# Autodesk Inventor assembly: BG201_trajan20_21
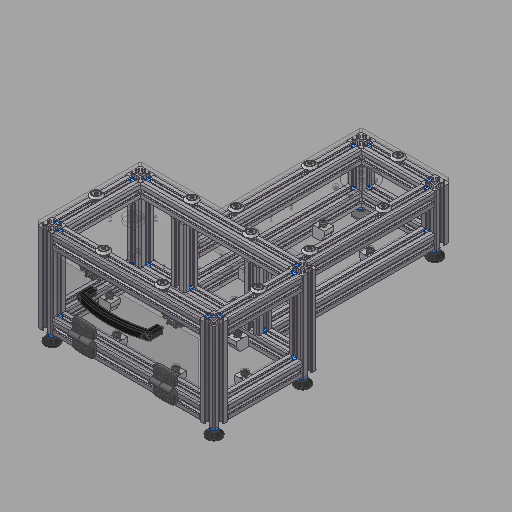
[picture p0: Inventor's stored thumbnail of the model, 512x512]
Saved by Autodesk Inventor 2022.2 (Build 262287000, 287)
## iProperties
Company: HTBLA Kaindorf
RuleStatus: InUse
Created: 2022-08-22
Part Number: BG201_trajan20_21
Project: Zeichenmaschine_v2
Material: Generisch
Description: gerüst_mit_platten
Document SubType Name: Assembly
Designer: trajan20
AfterDocNew0: iProperties-Editor_aufrufen
Author: jan
Keywords: 2021
## Documents named in this file (15)
- C:\Users\jan\Documents\DrawMachine\DrawMachineConstruction\Projekt\Zeichenmaschine_v2\BG201_trajan20_21_Zeichenmaschine_v2_gerüst_mit_platten.iam
- C:\Users\jan\Documents\DrawMachine\DrawMachineConstruction\Projekt\Zeichenmaschine_v2\BG103_trajan20_21_Zeichenmaschine_v2_Gerüst_Step_zu_Bauteil.iam
- C:\Users\jan\Documents\DrawMachine\DrawMachineConstruction\Projekt\Zeichenmaschine_v2\BT201_trajan20_21_Zeichenmaschine_v2_Hauptplatte unten.ipt
- C:\Users\jan\Documents\DrawMachine\DrawMachineConstruction\Projekt\Zeichenmaschine_v2\BT202_trajan20_21_Zeichenmaschine_v2_getriebemotor platte unten.ipt
- C:\Users\jan\Documents\DrawMachine\DrawMachineConstruction\Projekt\Zeichenmaschine_v2\BT101_trajan20_21_Zeichenmaschine_v2_Platte Stepper Motoren.ipt
- C:\Users\jan\Documents\DrawMachine\DrawMachineConstruction\Projekt\Zeichenmaschine_v2\BT102_trajan20_21_Zeichenmaschine_v2_Platte Getriebemotor.ipt
- C:\Users\jan\Documents\DrawMachine\DrawMachineConstruction\Projekt\Zeichenmaschine_v2\Normteile\de-DE\ISO 14583\ISO 14583 - M4x12-A3-70.ipt
- C:\Users\jan\Documents\DrawMachine\DrawMachineConstruction\Projekt\Zeichenmaschine_v2\step dateien\BN 603 1229915 finishing washer M5.ipt
- C:\Users\jan\Documents\DrawMachine\DrawMachineConstruction\Projekt\Zeichenmaschine_v2\Senkschraube DIN ≈965 M5x14 51305_050_014(High).ipt
- C:\Users\jan\Documents\DrawMachine\DrawMachineConstruction\Projekt\Zeichenmaschine_v2\ART 48240 - DIN 6900-1 Z0 T M4x12_0 mm - A2_Steel.ipt
- C:\Users\jan\Documents\DrawMachine\DrawMachineConstruction\Projekt\Zeichenmaschine_v2\Senkschraube DIN ≈965 M4x8 51305_040_008(High).ipt
- C:\Users\jan\Documents\DrawMachine\DrawMachineConstruction\Projekt\Zeichenmaschine_v2\BT703_trajan20_21_Zeichenmaschine_v2_Plexitür_200x80.ipt
- C:\Users\jan\Documents\DrawMachine\DrawMachineConstruction\Projekt\Zeichenmaschine_v2\Normteile\de-DE\AS 1427(03)\AS 1427 - M2 x 4(1).ipt
- C:\Users\jan\Documents\DrawMachine\DrawMachineConstruction\Projekt\Zeichenmaschine_v2\Normteile\de-DE\ISO 4762(2)\ISO 4762 - M4 x 16ISO.ipt
- C:\Users\jan\Documents\DrawMachine\DrawMachineConstruction\Projekt\Zeichenmaschine_v2\BT703_B_trajan20_21_Zeichenmaschine_v2_Griff.ipt
## Components (57 placed, 14 different names)
1. BG103_trajan20_21_Zeichenmaschine_v2_Gerüst_Step_zu_Bauteil:1 [sub-assembly] — Passend:1, Passend:2, Passend:3, Passend:4, Passend:5, Passend:6, Passend:7, Fluchtend:1, Fluchtend:2, Fluchtend:3, Passend:8, Fluchtend:4, Passend:64, Passend:65, Passend:66, Passend:67, Passend:68, Passend:69, Passend:70, Passend:71, Passend:72, Passend:73, Passend:74, Passend:75, Passend:76, Passend:77, Passend:78, Passend:79, Passend:83, Passend:85, Passend:86, Passend:87, Passend:88, Passend:89, Passend:90, Passend:91, Passend:92, Passend:93, Passend:94
2. BT201_trajan20_21_Zeichenmaschine_v2_Hauptplatte unten:1 — Passend:1, Passend:2, Passend:3, Einfügen:1, Passend:9, Passend:10, Passend:11, Passend:12, Passend:13, Passend:14, Passend:15, Passend:16, Passend:17, Passend:18
3. BT202_trajan20_21_Zeichenmaschine_v2_getriebemotor platte unten:1 — Passend:4, Passend:5, Passend:6, Passend:19, Passend:20, Passend:21, Passend:22, Passend:23, Passend:24, Passend:25, Passend:26, Passend:27, Passend:28, Passend:51, Passend:52
4. BT101_trajan20_21_Zeichenmaschine_v2_Platte Stepper Motoren:1 — Passend:7, Fluchtend:1, Fluchtend:2, Passend:29, Passend:30, Passend:31, Passend:32, Passend:33, Passend:34, Passend:35, Passend:36, Passend:37, Passend:38, Passend:39, Passend:40
5. BT102_trajan20_21_Zeichenmaschine_v2_Platte Getriebemotor:1 — Fluchtend:3, Passend:8, Fluchtend:4, Passend:41, Passend:42, Passend:43, Passend:44, Passend:45, Passend:46, Passend:47, Passend:48, Passend:49, Passend:50
6. BN 603 1229915 finishing washer M5:1 — Passend:29, Passend:30, Passend:62, Fluchtend:14
7. BN 603 1229915 finishing washer M5:2 — Passend:31, Passend:32, Passend:61, Fluchtend:13
8. BN 603 1229915 finishing washer M5:3 — Passend:33, Passend:34, Passend:60, Fluchtend:12
9. BN 603 1229915 finishing washer M5:4 — Passend:35, Passend:36, Passend:59, Fluchtend:11
10. BN 603 1229915 finishing washer M5:5 — Passend:37, Passend:38, Passend:58, Fluchtend:10
11. BN 603 1229915 finishing washer M5:6 — Passend:39, Passend:40, Passend:63, Fluchtend:15
12. BN 603 1229915 finishing washer M5:7 — Passend:41, Passend:42, Passend:54, Fluchtend:6
13. BN 603 1229915 finishing washer M5:8 — Passend:43, Passend:44, Passend:53, Fluchtend:5
14. BN 603 1229915 finishing washer M5:9 — Passend:45, Passend:46, Passend:57, Fluchtend:9
15. BN 603 1229915 finishing washer M5:10 — Passend:47, Passend:48, Passend:56, Fluchtend:8
16. BN 603 1229915 finishing washer M5:11 — Passend:49, Passend:50, Passend:55, Fluchtend:7
17. Schraube ISO 14583:2011(E) M4x12-A3-70:12 — Passend:51, Passend:52
18. Senkschraube DIN ≈965 M5x14 51305_050_014(High):1 — Passend:53, Fluchtend:5
19. Senkschraube DIN ≈965 M5x14 51305_050_014(High):2 — Passend:54, Fluchtend:6
20. Senkschraube DIN ≈965 M5x14 51305_050_014(High):3 — Passend:55, Fluchtend:7
21. Senkschraube DIN ≈965 M5x14 51305_050_014(High):4 — Passend:56, Fluchtend:8
22. Senkschraube DIN ≈965 M5x14 51305_050_014(High):5 — Passend:57, Fluchtend:9
23. Senkschraube DIN ≈965 M5x14 51305_050_014(High):6 — Passend:58, Fluchtend:10
24. Senkschraube DIN ≈965 M5x14 51305_050_014(High):7 — Passend:59, Fluchtend:11
25. Senkschraube DIN ≈965 M5x14 51305_050_014(High):8 — Passend:60, Fluchtend:12
26. Senkschraube DIN ≈965 M5x14 51305_050_014(High):9 — Passend:61, Fluchtend:13
27. Senkschraube DIN ≈965 M5x14 51305_050_014(High):10 — Passend:62, Fluchtend:14
28. Senkschraube DIN ≈965 M5x14 51305_050_014(High):11 — Passend:63, Fluchtend:15
29. ART 48240 - DIN 6900-1 Z0 T M4x12_0 mm - A2_Steel:1 — Passend:64, Passend:65
30. ART 48240 - DIN 6900-1 Z0 T M4x12_0 mm - A2_Steel:2 — Passend:66, Passend:67
31. ART 48240 - DIN 6900-1 Z0 T M4x12_0 mm - A2_Steel:3 — Passend:68, Passend:71
32. ART 48240 - DIN 6900-1 Z0 T M4x12_0 mm - A2_Steel:4 — Passend:69, Passend:70
33. Senkschraube DIN ≈965 M4x8 51305_040_008(High):1 — Passend:72, Passend:73
34. Senkschraube DIN ≈965 M4x8 51305_040_008(High):2 — Passend:74, Passend:75
35. Senkschraube DIN ≈965 M4x8 51305_040_008(High):3 — Passend:76, Passend:77
36. Senkschraube DIN ≈965 M4x8 51305_040_008(High):4 — Passend:78, Passend:79
37. BT703_trajan20_21_Zeichenmaschine_v2_Plexitür_200x80:1 — Passend:80, Passend:81, Passend:82, Passend:83, Passend:84, Passend:85, Passend:86, Passend:95, Passend:96, Passend:97
38. AS 1427 - Metrisch M2 x 4:1 — Passend:80, Passend:81
39. AS 1427 - Metrisch M2 x 4:2 — Passend:82, Passend:84
40. Senkschraube DIN ≈965 M4x8 51305_040_008(High):5 — Passend:87, Passend:93
41. Senkschraube DIN ≈965 M4x8 51305_040_008(High):6 — Passend:88, Passend:94
42. Senkschraube DIN ≈965 M4x8 51305_040_008(High):7 — Passend:89, Passend:92
43. Senkschraube DIN ≈965 M4x8 51305_040_008(High):8 — Passend:90, Passend:91
44. ISO 4762 M4 x 16:1 — Passend:98, Passend:101
45. BT703_B_trajan20_21_Zeichenmaschine_v2_Griff:1 — Passend:95, Passend:96, Passend:97, Passend:98, Passend:99, Passend:100, Passend:101
46. ISO 4762 M4 x 16:2 — Passend:99, Passend:100
47. Schraube ISO 14583:2011(E) M4x12-A3-70:1 — Einfügen:1
48. Schraube ISO 14583:2011(E) M4x12-A3-70:2 — Passend:9, Passend:10
49. Schraube ISO 14583:2011(E) M4x12-A3-70:3 — Passend:11, Passend:12
50. Schraube ISO 14583:2011(E) M4x12-A3-70:4 — Passend:13, Passend:14
51. Schraube ISO 14583:2011(E) M4x12-A3-70:5 — Passend:15, Passend:16
52. Schraube ISO 14583:2011(E) M4x12-A3-70:6 — Passend:17, Passend:18
53. Schraube ISO 14583:2011(E) M4x12-A3-70:7 — Passend:19, Passend:20
54. Schraube ISO 14583:2011(E) M4x12-A3-70:8 — Passend:21, Passend:22
55. Schraube ISO 14583:2011(E) M4x12-A3-70:9 — Passend:23, Passend:24
56. Schraube ISO 14583:2011(E) M4x12-A3-70:10 — Passend:25, Passend:26
57. Schraube ISO 14583:2011(E) M4x12-A3-70:11 — Passend:27, Passend:28
## Relationships (117: Mate 101, Flush 15, Insert 1)
- Passend:1 [Mate]: BG103_trajan20_21_Zeichenmaschine_v2_Gerüst_Step_zu_Bauteil:1 ↔ BT201_trajan20_21_Zeichenmaschine_v2_Hauptplatte unten:1
- Passend:2 [Mate]: BG103_trajan20_21_Zeichenmaschine_v2_Gerüst_Step_zu_Bauteil:1 ↔ BT201_trajan20_21_Zeichenmaschine_v2_Hauptplatte unten:1
- Passend:3 [Mate]: BG103_trajan20_21_Zeichenmaschine_v2_Gerüst_Step_zu_Bauteil:1 ↔ BT201_trajan20_21_Zeichenmaschine_v2_Hauptplatte unten:1
- Passend:4 [Mate]: BG103_trajan20_21_Zeichenmaschine_v2_Gerüst_Step_zu_Bauteil:1 ↔ BT202_trajan20_21_Zeichenmaschine_v2_getriebemotor platte unten:1
- Passend:5 [Mate]: BG103_trajan20_21_Zeichenmaschine_v2_Gerüst_Step_zu_Bauteil:1 ↔ BT202_trajan20_21_Zeichenmaschine_v2_getriebemotor platte unten:1
- Passend:6 [Mate]: BG103_trajan20_21_Zeichenmaschine_v2_Gerüst_Step_zu_Bauteil:1 ↔ BT202_trajan20_21_Zeichenmaschine_v2_getriebemotor platte unten:1
- Passend:7 [Mate]: BG103_trajan20_21_Zeichenmaschine_v2_Gerüst_Step_zu_Bauteil:1 ↔ BT101_trajan20_21_Zeichenmaschine_v2_Platte Stepper Motoren:1
- Fluchtend:1 [Flush]: BG103_trajan20_21_Zeichenmaschine_v2_Gerüst_Step_zu_Bauteil:1 ↔ BT101_trajan20_21_Zeichenmaschine_v2_Platte Stepper Motoren:1
- Fluchtend:2 [Flush]: BG103_trajan20_21_Zeichenmaschine_v2_Gerüst_Step_zu_Bauteil:1 ↔ BT101_trajan20_21_Zeichenmaschine_v2_Platte Stepper Motoren:1
- Fluchtend:3 [Flush]: BG103_trajan20_21_Zeichenmaschine_v2_Gerüst_Step_zu_Bauteil:1 ↔ BT102_trajan20_21_Zeichenmaschine_v2_Platte Getriebemotor:1
- Passend:8 [Mate]: BG103_trajan20_21_Zeichenmaschine_v2_Gerüst_Step_zu_Bauteil:1 ↔ BT102_trajan20_21_Zeichenmaschine_v2_Platte Getriebemotor:1
- Fluchtend:4 [Flush]: BG103_trajan20_21_Zeichenmaschine_v2_Gerüst_Step_zu_Bauteil:1 ↔ BT102_trajan20_21_Zeichenmaschine_v2_Platte Getriebemotor:1
- Einfügen:1 [Insert]: BT201_trajan20_21_Zeichenmaschine_v2_Hauptplatte unten:1 ↔ Schraube ISO 14583:2011(E) M4x12-A3-70:1
- Passend:9 [Mate]: BT201_trajan20_21_Zeichenmaschine_v2_Hauptplatte unten:1 ↔ Schraube ISO 14583:2011(E) M4x12-A3-70:2
- Passend:10 [Mate]: BT201_trajan20_21_Zeichenmaschine_v2_Hauptplatte unten:1 ↔ Schraube ISO 14583:2011(E) M4x12-A3-70:2
- Passend:11 [Mate]: BT201_trajan20_21_Zeichenmaschine_v2_Hauptplatte unten:1 ↔ Schraube ISO 14583:2011(E) M4x12-A3-70:3
- Passend:12 [Mate]: BT201_trajan20_21_Zeichenmaschine_v2_Hauptplatte unten:1 ↔ Schraube ISO 14583:2011(E) M4x12-A3-70:3
- Passend:13 [Mate]: BT201_trajan20_21_Zeichenmaschine_v2_Hauptplatte unten:1 ↔ Schraube ISO 14583:2011(E) M4x12-A3-70:4
- Passend:14 [Mate]: BT201_trajan20_21_Zeichenmaschine_v2_Hauptplatte unten:1 ↔ Schraube ISO 14583:2011(E) M4x12-A3-70:4
- Passend:15 [Mate]: BT201_trajan20_21_Zeichenmaschine_v2_Hauptplatte unten:1 ↔ Schraube ISO 14583:2011(E) M4x12-A3-70:5
- Passend:16 [Mate]: BT201_trajan20_21_Zeichenmaschine_v2_Hauptplatte unten:1 ↔ Schraube ISO 14583:2011(E) M4x12-A3-70:5
- Passend:17 [Mate]: BT201_trajan20_21_Zeichenmaschine_v2_Hauptplatte unten:1 ↔ Schraube ISO 14583:2011(E) M4x12-A3-70:6
- Passend:18 [Mate]: BT201_trajan20_21_Zeichenmaschine_v2_Hauptplatte unten:1 ↔ Schraube ISO 14583:2011(E) M4x12-A3-70:6
- Passend:19 [Mate]: BT202_trajan20_21_Zeichenmaschine_v2_getriebemotor platte unten:1 ↔ Schraube ISO 14583:2011(E) M4x12-A3-70:7
- Passend:20 [Mate]: BT202_trajan20_21_Zeichenmaschine_v2_getriebemotor platte unten:1 ↔ Schraube ISO 14583:2011(E) M4x12-A3-70:7
- Passend:21 [Mate]: BT202_trajan20_21_Zeichenmaschine_v2_getriebemotor platte unten:1 ↔ Schraube ISO 14583:2011(E) M4x12-A3-70:8
- Passend:22 [Mate]: BT202_trajan20_21_Zeichenmaschine_v2_getriebemotor platte unten:1 ↔ Schraube ISO 14583:2011(E) M4x12-A3-70:8
- Passend:23 [Mate]: BT202_trajan20_21_Zeichenmaschine_v2_getriebemotor platte unten:1 ↔ Schraube ISO 14583:2011(E) M4x12-A3-70:9
- Passend:24 [Mate]: BT202_trajan20_21_Zeichenmaschine_v2_getriebemotor platte unten:1 ↔ Schraube ISO 14583:2011(E) M4x12-A3-70:9
- Passend:25 [Mate]: BT202_trajan20_21_Zeichenmaschine_v2_getriebemotor platte unten:1 ↔ Schraube ISO 14583:2011(E) M4x12-A3-70:10
- Passend:26 [Mate]: BT202_trajan20_21_Zeichenmaschine_v2_getriebemotor platte unten:1 ↔ Schraube ISO 14583:2011(E) M4x12-A3-70:10
- Passend:27 [Mate]: BT202_trajan20_21_Zeichenmaschine_v2_getriebemotor platte unten:1 ↔ Schraube ISO 14583:2011(E) M4x12-A3-70:11
- Passend:28 [Mate]: BT202_trajan20_21_Zeichenmaschine_v2_getriebemotor platte unten:1 ↔ Schraube ISO 14583:2011(E) M4x12-A3-70:11
- Passend:29 [Mate]: BT101_trajan20_21_Zeichenmaschine_v2_Platte Stepper Motoren:1 ↔ BN 603 1229915 finishing washer M5:1
- Passend:30 [Mate]: BT101_trajan20_21_Zeichenmaschine_v2_Platte Stepper Motoren:1 ↔ BN 603 1229915 finishing washer M5:1
- Passend:31 [Mate]: BT101_trajan20_21_Zeichenmaschine_v2_Platte Stepper Motoren:1 ↔ BN 603 1229915 finishing washer M5:2
- Passend:32 [Mate]: BT101_trajan20_21_Zeichenmaschine_v2_Platte Stepper Motoren:1 ↔ BN 603 1229915 finishing washer M5:2
- Passend:33 [Mate]: BT101_trajan20_21_Zeichenmaschine_v2_Platte Stepper Motoren:1 ↔ BN 603 1229915 finishing washer M5:3
- Passend:34 [Mate]: BT101_trajan20_21_Zeichenmaschine_v2_Platte Stepper Motoren:1 ↔ BN 603 1229915 finishing washer M5:3
- Passend:35 [Mate]: BT101_trajan20_21_Zeichenmaschine_v2_Platte Stepper Motoren:1 ↔ BN 603 1229915 finishing washer M5:4
- Passend:36 [Mate]: BT101_trajan20_21_Zeichenmaschine_v2_Platte Stepper Motoren:1 ↔ BN 603 1229915 finishing washer M5:4
- Passend:37 [Mate]: BT101_trajan20_21_Zeichenmaschine_v2_Platte Stepper Motoren:1 ↔ BN 603 1229915 finishing washer M5:5
- Passend:38 [Mate]: BT101_trajan20_21_Zeichenmaschine_v2_Platte Stepper Motoren:1 ↔ BN 603 1229915 finishing washer M5:5
- Passend:39 [Mate]: BT101_trajan20_21_Zeichenmaschine_v2_Platte Stepper Motoren:1 ↔ BN 603 1229915 finishing washer M5:6
- Passend:40 [Mate]: BT101_trajan20_21_Zeichenmaschine_v2_Platte Stepper Motoren:1 ↔ BN 603 1229915 finishing washer M5:6
- Passend:41 [Mate]: BT102_trajan20_21_Zeichenmaschine_v2_Platte Getriebemotor:1 ↔ BN 603 1229915 finishing washer M5:7
- Passend:42 [Mate]: BT102_trajan20_21_Zeichenmaschine_v2_Platte Getriebemotor:1 ↔ BN 603 1229915 finishing washer M5:7
- Passend:43 [Mate]: BT102_trajan20_21_Zeichenmaschine_v2_Platte Getriebemotor:1 ↔ BN 603 1229915 finishing washer M5:8
- Passend:44 [Mate]: BT102_trajan20_21_Zeichenmaschine_v2_Platte Getriebemotor:1 ↔ BN 603 1229915 finishing washer M5:8
- Passend:45 [Mate]: BT102_trajan20_21_Zeichenmaschine_v2_Platte Getriebemotor:1 ↔ BN 603 1229915 finishing washer M5:9
- Passend:46 [Mate]: BT102_trajan20_21_Zeichenmaschine_v2_Platte Getriebemotor:1 ↔ BN 603 1229915 finishing washer M5:9
- Passend:47 [Mate]: BT102_trajan20_21_Zeichenmaschine_v2_Platte Getriebemotor:1 ↔ BN 603 1229915 finishing washer M5:10
- Passend:48 [Mate]: BT102_trajan20_21_Zeichenmaschine_v2_Platte Getriebemotor:1 ↔ BN 603 1229915 finishing washer M5:10
- Passend:49 [Mate]: BT102_trajan20_21_Zeichenmaschine_v2_Platte Getriebemotor:1 ↔ BN 603 1229915 finishing washer M5:11
- Passend:50 [Mate]: BT102_trajan20_21_Zeichenmaschine_v2_Platte Getriebemotor:1 ↔ BN 603 1229915 finishing washer M5:11
- Passend:51 [Mate]: BT202_trajan20_21_Zeichenmaschine_v2_getriebemotor platte unten:1 ↔ Schraube ISO 14583:2011(E) M4x12-A3-70:12
- Passend:52 [Mate]: BT202_trajan20_21_Zeichenmaschine_v2_getriebemotor platte unten:1 ↔ Schraube ISO 14583:2011(E) M4x12-A3-70:12
- Passend:53 [Mate]: BN 603 1229915 finishing washer M5:8 ↔ Senkschraube DIN ≈965 M5x14 51305_050_014(High):1
- Fluchtend:5 [Flush]: BN 603 1229915 finishing washer M5:8 ↔ Senkschraube DIN ≈965 M5x14 51305_050_014(High):1
- Passend:54 [Mate]: BN 603 1229915 finishing washer M5:7 ↔ Senkschraube DIN ≈965 M5x14 51305_050_014(High):2
- Fluchtend:6 [Flush]: BN 603 1229915 finishing washer M5:7 ↔ Senkschraube DIN ≈965 M5x14 51305_050_014(High):2
- Passend:55 [Mate]: BN 603 1229915 finishing washer M5:11 ↔ Senkschraube DIN ≈965 M5x14 51305_050_014(High):3
- Fluchtend:7 [Flush]: BN 603 1229915 finishing washer M5:11 ↔ Senkschraube DIN ≈965 M5x14 51305_050_014(High):3
- Passend:56 [Mate]: BN 603 1229915 finishing washer M5:10 ↔ Senkschraube DIN ≈965 M5x14 51305_050_014(High):4
- Fluchtend:8 [Flush]: BN 603 1229915 finishing washer M5:10 ↔ Senkschraube DIN ≈965 M5x14 51305_050_014(High):4
- Passend:57 [Mate]: BN 603 1229915 finishing washer M5:9 ↔ Senkschraube DIN ≈965 M5x14 51305_050_014(High):5
- Fluchtend:9 [Flush]: BN 603 1229915 finishing washer M5:9 ↔ Senkschraube DIN ≈965 M5x14 51305_050_014(High):5
- Passend:58 [Mate]: BN 603 1229915 finishing washer M5:5 ↔ Senkschraube DIN ≈965 M5x14 51305_050_014(High):6
- Fluchtend:10 [Flush]: BN 603 1229915 finishing washer M5:5 ↔ Senkschraube DIN ≈965 M5x14 51305_050_014(High):6
- Passend:59 [Mate]: BN 603 1229915 finishing washer M5:4 ↔ Senkschraube DIN ≈965 M5x14 51305_050_014(High):7
- Fluchtend:11 [Flush]: BN 603 1229915 finishing washer M5:4 ↔ Senkschraube DIN ≈965 M5x14 51305_050_014(High):7
- Passend:60 [Mate]: BN 603 1229915 finishing washer M5:3 ↔ Senkschraube DIN ≈965 M5x14 51305_050_014(High):8
- Fluchtend:12 [Flush]: BN 603 1229915 finishing washer M5:3 ↔ Senkschraube DIN ≈965 M5x14 51305_050_014(High):8
- Passend:61 [Mate]: BN 603 1229915 finishing washer M5:2 ↔ Senkschraube DIN ≈965 M5x14 51305_050_014(High):9
- Fluchtend:13 [Flush]: BN 603 1229915 finishing washer M5:2 ↔ Senkschraube DIN ≈965 M5x14 51305_050_014(High):9
- Passend:62 [Mate]: BN 603 1229915 finishing washer M5:1 ↔ Senkschraube DIN ≈965 M5x14 51305_050_014(High):10
- Fluchtend:14 [Flush]: BN 603 1229915 finishing washer M5:1 ↔ Senkschraube DIN ≈965 M5x14 51305_050_014(High):10
- Passend:63 [Mate]: BN 603 1229915 finishing washer M5:6 ↔ Senkschraube DIN ≈965 M5x14 51305_050_014(High):11
- Fluchtend:15 [Flush]: BN 603 1229915 finishing washer M5:6 ↔ Senkschraube DIN ≈965 M5x14 51305_050_014(High):11
- Passend:64 [Mate]: BG103_trajan20_21_Zeichenmaschine_v2_Gerüst_Step_zu_Bauteil:1 ↔ ART 48240 - DIN 6900-1 Z0 T M4x12_0 mm - A2_Steel:1
- Passend:65 [Mate]: BG103_trajan20_21_Zeichenmaschine_v2_Gerüst_Step_zu_Bauteil:1 ↔ ART 48240 - DIN 6900-1 Z0 T M4x12_0 mm - A2_Steel:1
- Passend:66 [Mate]: BG103_trajan20_21_Zeichenmaschine_v2_Gerüst_Step_zu_Bauteil:1 ↔ ART 48240 - DIN 6900-1 Z0 T M4x12_0 mm - A2_Steel:2
- Passend:67 [Mate]: BG103_trajan20_21_Zeichenmaschine_v2_Gerüst_Step_zu_Bauteil:1 ↔ ART 48240 - DIN 6900-1 Z0 T M4x12_0 mm - A2_Steel:2
- Passend:68 [Mate]: BG103_trajan20_21_Zeichenmaschine_v2_Gerüst_Step_zu_Bauteil:1 ↔ ART 48240 - DIN 6900-1 Z0 T M4x12_0 mm - A2_Steel:3
- Passend:69 [Mate]: BG103_trajan20_21_Zeichenmaschine_v2_Gerüst_Step_zu_Bauteil:1 ↔ ART 48240 - DIN 6900-1 Z0 T M4x12_0 mm - A2_Steel:4
- Passend:70 [Mate]: BG103_trajan20_21_Zeichenmaschine_v2_Gerüst_Step_zu_Bauteil:1 ↔ ART 48240 - DIN 6900-1 Z0 T M4x12_0 mm - A2_Steel:4
- Passend:71 [Mate]: BG103_trajan20_21_Zeichenmaschine_v2_Gerüst_Step_zu_Bauteil:1 ↔ ART 48240 - DIN 6900-1 Z0 T M4x12_0 mm - A2_Steel:3
- Passend:72 [Mate]: BG103_trajan20_21_Zeichenmaschine_v2_Gerüst_Step_zu_Bauteil:1 ↔ Senkschraube DIN ≈965 M4x8 51305_040_008(High):1
- Passend:73 [Mate]: BG103_trajan20_21_Zeichenmaschine_v2_Gerüst_Step_zu_Bauteil:1 ↔ Senkschraube DIN ≈965 M4x8 51305_040_008(High):1
- Passend:74 [Mate]: BG103_trajan20_21_Zeichenmaschine_v2_Gerüst_Step_zu_Bauteil:1 ↔ Senkschraube DIN ≈965 M4x8 51305_040_008(High):2
- Passend:75 [Mate]: BG103_trajan20_21_Zeichenmaschine_v2_Gerüst_Step_zu_Bauteil:1 ↔ Senkschraube DIN ≈965 M4x8 51305_040_008(High):2
- Passend:76 [Mate]: BG103_trajan20_21_Zeichenmaschine_v2_Gerüst_Step_zu_Bauteil:1 ↔ Senkschraube DIN ≈965 M4x8 51305_040_008(High):3
- Passend:77 [Mate]: BG103_trajan20_21_Zeichenmaschine_v2_Gerüst_Step_zu_Bauteil:1 ↔ Senkschraube DIN ≈965 M4x8 51305_040_008(High):3
- Passend:78 [Mate]: BG103_trajan20_21_Zeichenmaschine_v2_Gerüst_Step_zu_Bauteil:1 ↔ Senkschraube DIN ≈965 M4x8 51305_040_008(High):4
- Passend:79 [Mate]: BG103_trajan20_21_Zeichenmaschine_v2_Gerüst_Step_zu_Bauteil:1 ↔ Senkschraube DIN ≈965 M4x8 51305_040_008(High):4
- Passend:80 [Mate]: BT703_trajan20_21_Zeichenmaschine_v2_Plexitür_200x80:1 ↔ AS 1427 - Metrisch M2 x 4:1
- Passend:81 [Mate]: BT703_trajan20_21_Zeichenmaschine_v2_Plexitür_200x80:1 ↔ AS 1427 - Metrisch M2 x 4:1
- Passend:82 [Mate]: BT703_trajan20_21_Zeichenmaschine_v2_Plexitür_200x80:1 ↔ AS 1427 - Metrisch M2 x 4:2
- Passend:83 [Mate]: BG103_trajan20_21_Zeichenmaschine_v2_Gerüst_Step_zu_Bauteil:1 ↔ BT703_trajan20_21_Zeichenmaschine_v2_Plexitür_200x80:1
- Passend:84 [Mate]: BT703_trajan20_21_Zeichenmaschine_v2_Plexitür_200x80:1 ↔ AS 1427 - Metrisch M2 x 4:2
- Passend:85 [Mate]: BG103_trajan20_21_Zeichenmaschine_v2_Gerüst_Step_zu_Bauteil:1 ↔ BT703_trajan20_21_Zeichenmaschine_v2_Plexitür_200x80:1
- Passend:86 [Mate]: BG103_trajan20_21_Zeichenmaschine_v2_Gerüst_Step_zu_Bauteil:1 ↔ BT703_trajan20_21_Zeichenmaschine_v2_Plexitür_200x80:1
- Passend:87 [Mate]: BG103_trajan20_21_Zeichenmaschine_v2_Gerüst_Step_zu_Bauteil:1 ↔ Senkschraube DIN ≈965 M4x8 51305_040_008(High):5
- Passend:88 [Mate]: BG103_trajan20_21_Zeichenmaschine_v2_Gerüst_Step_zu_Bauteil:1 ↔ Senkschraube DIN ≈965 M4x8 51305_040_008(High):6
- Passend:89 [Mate]: BG103_trajan20_21_Zeichenmaschine_v2_Gerüst_Step_zu_Bauteil:1 ↔ Senkschraube DIN ≈965 M4x8 51305_040_008(High):7
- Passend:90 [Mate]: BG103_trajan20_21_Zeichenmaschine_v2_Gerüst_Step_zu_Bauteil:1 ↔ Senkschraube DIN ≈965 M4x8 51305_040_008(High):8
- Passend:91 [Mate]: BG103_trajan20_21_Zeichenmaschine_v2_Gerüst_Step_zu_Bauteil:1 ↔ Senkschraube DIN ≈965 M4x8 51305_040_008(High):8
- Passend:92 [Mate]: BG103_trajan20_21_Zeichenmaschine_v2_Gerüst_Step_zu_Bauteil:1 ↔ Senkschraube DIN ≈965 M4x8 51305_040_008(High):7
- Passend:93 [Mate]: BG103_trajan20_21_Zeichenmaschine_v2_Gerüst_Step_zu_Bauteil:1 ↔ Senkschraube DIN ≈965 M4x8 51305_040_008(High):5
- Passend:94 [Mate]: BG103_trajan20_21_Zeichenmaschine_v2_Gerüst_Step_zu_Bauteil:1 ↔ Senkschraube DIN ≈965 M4x8 51305_040_008(High):6
- Passend:95 [Mate]: BT703_trajan20_21_Zeichenmaschine_v2_Plexitür_200x80:1 ↔ BT703_B_trajan20_21_Zeichenmaschine_v2_Griff:1
- Passend:96 [Mate]: BT703_trajan20_21_Zeichenmaschine_v2_Plexitür_200x80:1 ↔ BT703_B_trajan20_21_Zeichenmaschine_v2_Griff:1
- Passend:97 [Mate]: BT703_trajan20_21_Zeichenmaschine_v2_Plexitür_200x80:1 ↔ BT703_B_trajan20_21_Zeichenmaschine_v2_Griff:1
- Passend:98 [Mate]: ISO 4762 M4 x 16:1 ↔ BT703_B_trajan20_21_Zeichenmaschine_v2_Griff:1
- Passend:99 [Mate]: BT703_B_trajan20_21_Zeichenmaschine_v2_Griff:1 ↔ ISO 4762 M4 x 16:2
- Passend:100 [Mate]: BT703_B_trajan20_21_Zeichenmaschine_v2_Griff:1 ↔ ISO 4762 M4 x 16:2
- Passend:101 [Mate]: ISO 4762 M4 x 16:1 ↔ BT703_B_trajan20_21_Zeichenmaschine_v2_Griff:1
